# Autodesk Inventor assembly: Transmission w 5 inch shaft and bracket assembly
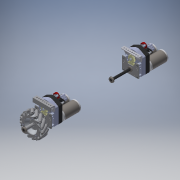
[picture p0: Inventor's stored thumbnail of the model, 180x180]
Saved by Autodesk Inventor 2016 SP2 (Build 200236200, 236)
## iProperties
Created: 2018-02-04
Part Number: Transmission w 5 inch shaft and bracket assembly
Document SubType Name: Assembly
Designer: CAD
Author: CAD
## Documents named in this file (6)
- C:\Users\CAD\Documents\GitHub\FIRST-ROBOTICS-2018-5436-CAD\Robot\Chassis\Transmission parts\Transmission w 5 inch shaft and bracket assembly.iam
- C:\Users\CAD\Desktop\new transmission layout 2.4.18.iam
- C:\Users\CAD\Documents\GitHub\FIRST-ROBOTICS-2018-5436-CAD\Robot\Chassis\wheels\am-3479R+6+SR+Mecanum+Right.iam
- C:\Users\CAD\Documents\GitHub\FIRST-ROBOTICS-2018-5436-CAD\Robot\Chassis\PVC spacers.ipt
- C:\Users\CAD\Documents\GitHub\FIRST-ROBOTICS-2018-5436-CAD\Robot\Chassis\PVC spacers 2in.ipt
- C:\Users\CAD\Documents\GitHub\FIRST-ROBOTICS-2018-5436-CAD\Robot\Chassis\4 L aluminum piece for transmission bracket.ipt
## Components (6 placed, 5 different names)
1. new transmission layout 2.4.18:2 [sub-assembly] — Mate:1, Mate:2, Mate:3, Mate:4, Mate:5, Mate:6
2. am-3479R+6+SR+Mecanum+Right:1 [sub-assembly] — Mate:1, Mate:2, Mate:3
3. PVC spacers:1
4. PVC spacers 2in:1
5. new transmission layout 2.4.18:3 [sub-assembly]
6. 4 L aluminum piece for transmission bracket:1 — Mate:4, Mate:5, Mate:6
## Relationships (6: Mate 6)
- Mate:1 (38.1 mm): new transmission layout 2.4.18:2 ↔ am-3479R+6+SR+Mecanum+Right:1
- Mate:2: new transmission layout 2.4.18:2 ↔ am-3479R+6+SR+Mecanum+Right:1
- Mate:3: new transmission layout 2.4.18:2 ↔ am-3479R+6+SR+Mecanum+Right:1
- Mate:4: new transmission layout 2.4.18:2 ↔ 4 L aluminum piece for transmission bracket:1
- Mate:5: new transmission layout 2.4.18:2 ↔ 4 L aluminum piece for transmission bracket:1
- Mate:6: new transmission layout 2.4.18:2 ↔ 4 L aluminum piece for transmission bracket:1
